# Autodesk Inventor assembly: bec
Saved by Autodesk Inventor 2021 (Build 250183000, 183)
## iProperties
Created: 2021-01-23
Part Number: bec
Document SubType Name: Assembly
Designer: User
Author: User
## Documents named in this file (10)
- D:\SynologyDrive\tcodev\tco-cad\common\bec\bec.iam
- D:\SynologyDrive\tcodev\tco-cad\common\bec\board.ipt
- D:\SynologyDrive\tcodev\tco-cad\common\kicad_packages_3d\PinHeader_1x06_P2.54mm_Vertical.ipt
- D:\SynologyDrive\tcodev\tco-cad\common\bec\heatsink.ipt
- D:\SynologyDrive\tcodev\tco-cad\common\kicad_packages_3d\L_Bourns_SRR1260.ipt
- D:\SynologyDrive\tcodev\tco-cad\common\kicad_packages_3d\TO-263-2.ipt
- D:\SynologyDrive\tcodev\tco-cad\common\kicad_packages_3d\TO-252-2.ipt
- D:\SynologyDrive\tcodev\tco-cad\common\kicad_packages_3d\C_Radial_D8.0mm_H11.5mm_P3.50mm.ipt
- D:\SynologyDrive\tcodev\tco-cad\common\kicad_packages_3d\C_Radial_D10.0mm_H20.0mm_P5.00mm.ipt
- D:\SynologyDrive\tcodev\tco-cad\common\samtec_parts\snt_100_bk_h_h\SNT-100-BK-H-H.iam
## Components (10 placed, 9 different names)
1. board:1 — Mate:1, Flush:1, Flush:2, Mate:2, Flush:3, Flush:4, Mate:3, Mate:4, Mate:5, Angle:1, Angle:2, Angle:3, Tangent:2, Flush:7, Tangent:3, Tangent:4, Flush:8
2. PinHeader_1x06_P2.54mm_Vertical:1 — Mate:1, Flush:1, Flush:2, Mate:7, Mate:8, Mate:9
3. heatsink:1
4. L_Bourns_SRR1260:1 — Mate:2, Flush:3, Flush:4, Mate:6
5. TO-263-2:1 — Mate:3, Angle:1
6. TO-252-2:1 — Mate:5, Angle:3, Flush:5
7. TO-252-2:2 — Mate:4, Angle:2, Flush:5
8. C_Radial_D10.0mm_H20.0mm_P5.00mm:1 — Tangent:2, Flush:7, Tangent:3
9. C_Radial_D8.0mm_H11.5mm_P3.50mm:1 — Tangent:4, Flush:8, Mate:6
10. SNT-100-BK-H-H:1 [sub-assembly] — Mate:7, Mate:8, Mate:9
## Relationships (22: Mate 9, Flush 7, Angle 3, Tangent 3)
- Mate:1 (-0.95 mm): board:1 ↔ PinHeader_1x06_P2.54mm_Vertical:1
- Flush:1 (4.88 mm): board:1 ↔ PinHeader_1x06_P2.54mm_Vertical:1
- Flush:2 (-2.54 mm): board:1 ↔ PinHeader_1x06_P2.54mm_Vertical:1
- Mate:2: board:1 ↔ L_Bourns_SRR1260:1
- Flush:3 (17 mm): board:1 ↔ L_Bourns_SRR1260:1
- Flush:4: board:1 ↔ L_Bourns_SRR1260:1
- Mate:3: board:1 ↔ TO-263-2:1
- Mate:4: board:1 ↔ TO-252-2:2
- Mate:5: board:1 ↔ TO-252-2:1
- Angle:1 (0 deg): board:1 ↔ TO-263-2:1
- Angle:2 (0 deg): board:1 ↔ TO-252-2:2
- Angle:3 (0 deg): board:1 ↔ TO-252-2:1
- Flush:5: TO-252-2:1 ↔ TO-252-2:2
- Tangent:2: board:1 ↔ C_Radial_D10.0mm_H20.0mm_P5.00mm:1
- Flush:7 (2.6 mm): board:1 ↔ C_Radial_D10.0mm_H20.0mm_P5.00mm:1
- Tangent:3: board:1 ↔ C_Radial_D10.0mm_H20.0mm_P5.00mm:1
- Tangent:4: board:1 ↔ C_Radial_D8.0mm_H11.5mm_P3.50mm:1
- Flush:8 (6 mm): board:1 ↔ C_Radial_D8.0mm_H11.5mm_P3.50mm:1
- Mate:6 (6 mm): L_Bourns_SRR1260:1 ↔ C_Radial_D8.0mm_H11.5mm_P3.50mm:1
- Mate:7: PinHeader_1x06_P2.54mm_Vertical:1 ↔ SNT-100-BK-H-H:1
- Mate:8 (0.277 mm): PinHeader_1x06_P2.54mm_Vertical:1 ↔ SNT-100-BK-H-H:1
- Mate:9 (0.277 mm): PinHeader_1x06_P2.54mm_Vertical:1 ↔ SNT-100-BK-H-H:1
